# Autodesk Inventor assembly: Assemble_test
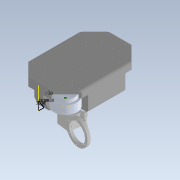
[picture p0: Inventor's stored thumbnail of the model, 180x180]
Saved by Autodesk Inventor 2020 (Build 240168000, 168)
## iProperties
Created: 2020-12-28
Part Number: Assemble_test
Document SubType Name: Assembly
Designer: DELL
Author: DELL
## Documents named in this file (6)
- F:\SoftRobot2.0\Flexipod2.0\robot_2020_12_28\Assemble_test.iam
- F:\SoftRobot2.0\Flexipod2.0\body\body_2020_12_28_13_34.ipt
- F:\SoftRobot2.0\Flexipod2.0\leg5_2020_12_24_11_46\hip_link_2.ipt
- F:\SoftRobot2.0\Flexipod2.0\RMD_X6_stator.ipt
- F:\SoftRobot2.0\Flexipod2.0\RMD_X6_rotor.ipt
- F:\SoftRobot2.0\Flexipod2.0\Arducam Camera.ipt
## Components (6 placed, 5 different names)
1. body_2020_12_28_13_34:1 — Mate:1, Mate:2, Mate:3, Mate:8, Angle:1, Mate:9, Mate:10, Mate:11, Angle:2
2. hip_link_2:1 — Mate:5, Mate:6, Mate:7
3. RMD_X6_stator:1 — Mate:1, Mate:2, Mate:3, Mate:4, Flush:1
4. RMD_X6_rotor:1 — Mate:4, Flush:1, Mate:5, Mate:6, Mate:7
5. Arducam Camera:1 — Mate:8, Angle:1, Mate:9
6. Arducam Camera:13 — Mate:10, Mate:11, Angle:2
## Relationships (14: Mate 11, Angle 2, Flush 1)
- Mate:1: body_2020_12_28_13_34:1 ↔ RMD_X6_stator:1
- Mate:2: body_2020_12_28_13_34:1 ↔ RMD_X6_stator:1
- Mate:3: body_2020_12_28_13_34:1 ↔ RMD_X6_stator:1
- Mate:4: RMD_X6_stator:1 ↔ RMD_X6_rotor:1
- Flush:1 (-3 mm): RMD_X6_stator:1 ↔ RMD_X6_rotor:1
- Mate:5: hip_link_2:1 ↔ RMD_X6_rotor:1
- Mate:6: hip_link_2:1 ↔ RMD_X6_rotor:1
- Mate:7: hip_link_2:1 ↔ RMD_X6_rotor:1
- Mate:8: body_2020_12_28_13_34:1 ↔ Arducam Camera:1
- Angle:1 (180 deg): body_2020_12_28_13_34:1 ↔ Arducam Camera:1
- Mate:9: body_2020_12_28_13_34:1 ↔ Arducam Camera:1
- Mate:10: body_2020_12_28_13_34:1 ↔ Arducam Camera:13
- Mate:11: body_2020_12_28_13_34:1 ↔ Arducam Camera:13
- Angle:2 (180 deg): body_2020_12_28_13_34:1 ↔ Arducam Camera:13
